# Autodesk Inventor assembly: A2017_T2_05
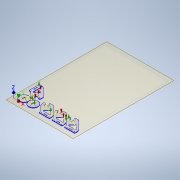
[picture p0: Inventor's stored thumbnail of the model, 180x180]
Saved by Autodesk Inventor 2020 (Build 240168000, 168)
## iProperties
Created: 2021-08-27
Part Number: A2017_T2_05
Document SubType Name: Assembly
Designer: Masato
Author: Masato
## Documents named in this file (4)
- C:\Users\marin\Documents\0118 git clone\OpenPlatform_ver3_0\cam\A2017_T2_05.iam
- C:\Users\marin\Documents\0118 git clone\OpenPlatform_ver3_0\cam\Disposable_Board.ipt
- C:\Users\marin\Documents\0118 git clone\OpenPlatform_ver3_0\UpperBody\Trunk\CrossRollerBearing\Inner_flange.ipt
- C:\Users\marin\Documents\0118 git clone\OpenPlatform_ver3_0\UpperBody\Arm\Shoulder_side_frame.ipt
## Components (7 placed, 3 different names)
1. Disposable_Board:1 — メイト:2, メイト:1, フラッシュ:1, フラッシュ:2, 正接:1, 正接:2, 角度:1, フラッシュ:3, フラッシュ:4, メイト:6, フラッシュ:5
2. Shoulder_side_frame:4 — メイト:6, フラッシュ:5, 正接:3
3. Inner_flange:1 — メイト:4, 正接:1, 正接:2, 角度:1, 正接:3
4. Inner_flange:2
5. Shoulder_side_frame:1 — メイト:5, フラッシュ:3, フラッシュ:4
6. Shoulder_side_frame:2
7. Shoulder_side_frame:3
## Component patterns: (2 elements, first: Inner_flange:1), (3 elements, first: Shoulder_side_frame:1)
## Relationships (14: Mate 5, Flush 5, Tangent 3, Angle 1)
- メイト:2 [Mate]: Disposable_Board:1
- メイト:1 [Mate]: Disposable_Board:1
- フラッシュ:1 [Flush]: Disposable_Board:1
- フラッシュ:2 [Flush]: Disposable_Board:1
- メイト:4 [Mate]: Inner_flange:1
- 正接:1 [Tangent] (3 mm): Disposable_Board:1 ↔ Inner_flange:1
- 正接:2 [Tangent] (3 mm): Disposable_Board:1 ↔ Inner_flange:1
- 角度:1 [Angle] (0 deg): Disposable_Board:1 ↔ Inner_flange:1
- メイト:5 [Mate]: Shoulder_side_frame:1
- フラッシュ:3 [Flush] (3 mm): Disposable_Board:1 ↔ Shoulder_side_frame:1
- フラッシュ:4 [Flush] (3 mm): Disposable_Board:1 ↔ Shoulder_side_frame:1
- メイト:6 [Mate]: Disposable_Board:1 ↔ Shoulder_side_frame:4
- フラッシュ:5 [Flush] (3 mm): Disposable_Board:1 ↔ Shoulder_side_frame:4
- 正接:3 [Tangent] (3.3 mm): Shoulder_side_frame:4 ↔ Inner_flange:1
